# Autodesk Inventor assembly: AM14U Long
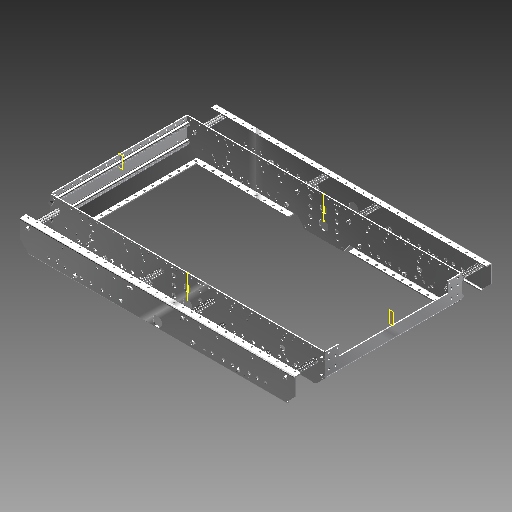
[picture p0: Inventor's stored thumbnail of the model, 512x512]
Saved by Autodesk Inventor 2017 (Build 210142000, 142)
## iProperties
Created: 2014-01-08
Part Number: AM14U Long
Document SubType Name: Assembly
Designer: 300593
Mass: 4367.68 g
Surface Area: 11268.2 cm^2
Volume: 1617.66 cm^3
Density: 2.7 g/cm^3
Author: 300593
## Documents named in this file (3)
- \\Mac\Home\Desktop\bunnybots 2016\15102898-16-Bunnybot-CAD\Bunnybot-To_be_renamed\15102898-16-A-0000\15102898-16-A-0100\AM14U Long.iam
- \\Mac\Home\Desktop\bunnybots 2016\15102898-16-Bunnybot-CAD\Bunnybot-To_be_renamed\15102898-16-A-0000\15102898-16-A-0100\AM14U Long Half.iam
- \\Mac\Home\Desktop\bunnybots 2016\15102898-16-Bunnybot-CAD\Bunnybot-To_be_renamed\15102898-16-A-0000\15102898-16-A-0100\Cross Brace Extrusion 15-75_CPY.ipt
## Components (3 placed, 2 different names)
1. AM14U Long Half:1 [sub-assembly] — Flush:2, Flush:3, Mate:2
2. AM14U Long Half:2 [sub-assembly] — Mate:1
3. Cross Brace Extrusion 15-75_CPY:1 — Mate:1, Flush:2, Flush:3, Mate:2
## Relationships (4: Mate 2, Flush 2)
- Mate:1: AM14U Long Half:2 ↔ Cross Brace Extrusion 15-75_CPY:1
- Flush:2: AM14U Long Half:1 ↔ Cross Brace Extrusion 15-75_CPY:1
- Flush:3: AM14U Long Half:1 ↔ Cross Brace Extrusion 15-75_CPY:1
- Mate:2: AM14U Long Half:1 ↔ Cross Brace Extrusion 15-75_CPY:1
